# Autodesk Inventor assembly: 二連趕
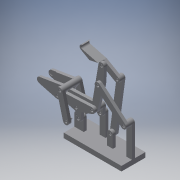
[picture p0: Inventor's stored thumbnail of the model, 180x180]
Saved by Autodesk Inventor 2017 (Build 210142000, 142)
## iProperties
Part Number: 二連趕
Material: 一般
Document SubType Name: Assembly
Designer: 士正
Author: 士正
## Documents named in this file (12)
- C:\Users\士正\Desktop\git\兩段式機構 Inventor版本\二連趕.iam
- C:\Users\士正\Desktop\git\兩段式機構 Inventor版本\實體2.ipt
- C:\Users\士正\Desktop\git\兩段式機構 Inventor版本\實體1.ipt
- C:\Users\士正\Desktop\git\兩段式機構 Inventor版本\實體3.ipt
- C:\Users\士正\Desktop\git\兩段式機構 Inventor版本\實體4.ipt
- C:\Users\士正\Desktop\git\兩段式機構 Inventor版本\實體5.ipt
- C:\Users\士正\Desktop\git\兩段式機構 Inventor版本\實體6.ipt
- C:\Users\士正\Desktop\git\兩段式機構 Inventor版本\實體7.ipt
- C:\Users\士正\Desktop\git\兩段式機構 Inventor版本\實體8.ipt
- C:\Users\士正\Desktop\git\兩段式機構 Inventor版本\實體9.ipt
- C:\Users\士正\Desktop\git\兩段式機構 Inventor版本\實體11.ipt
- C:\Users\士正\Desktop\git\兩段式機構 Inventor版本\pin.ipt
## Components (26 placed, 11 different names)
1. 實體2:1 — 貼合:6, 貼合:15, 貼合:26, 貼合:41, 齊平:11, 貼合:43, 齊平:13
2. 實體1:1 — 貼合:3, 貼合:8, 貼合:21, 貼合:39, 齊平:9, 貼合:60
3. 實體4:1 — 貼合:9, 貼合:11, 貼合:30, 貼合:31
4. 實體5:1 — 貼合:10, 貼合:11, 貼合:31, 貼合:35, 齊平:5
5. 實體6:1 — 貼合:4, 貼合:7, 貼合:33, 齊平:3, 貼合:47, 齊平:18
6. 實體9:1 — 貼合:7, 貼合:8, 貼合:10, 貼合:36, 齊平:6, 貼合:37, 貼合:47, 貼合:60, 貼合:70, 貼合:71
7. 實體11:1 — 貼合:1, 齊平:1, 齊平:2, 貼合:3, 貼合:4, 貼合:6, 貼合:9, 貼合:16, 貼合:21, 貼合:30, 貼合:34, 齊平:4, 貼合:48, 貼合:53, 貼合:58
8. 實體2:2 — 貼合:16, 貼合:53, 貼合:64, 齊平:20, 貼合:66, 貼合:67, 齊平:22, 貼合:68
9. 實體7:2 — 貼合:15, 貼合:26, 貼合:44, 齊平:14, 貼合:56, 貼合:65, 齊平:21, 貼合:66, 貼合:68, 貼合:69
10. pin:1 — 貼合:37, 齊平:18
11. pin:2 — 齊平:17, 貼合:72, 齊平:23
12. pin:3 — 貼合:36, 齊平:6
13. pin:5 — 貼合:67, 齊平:22
14. pin:6 — 貼合:49, 齊平:16
15. pin:7 — 貼合:41, 齊平:11
16. pin:8 — 貼合:35, 齊平:5
17. pin:9 — 貼合:34, 齊平:4
18. pin:10 — 貼合:33, 齊平:3
19. pin:11 — 貼合:39, 齊平:9
20. pin:12
21. pin:13 — 貼合:43, 齊平:13
22. pin:14 — 貼合:44, 齊平:14
23. 實體3:1 — 貼合:48, 貼合:49, 貼合:51, 貼合:55, 貼合:58
24. 實體8:1 — 貼合:51, 貼合:55, 貼合:56, 齊平:16, 齊平:17, 貼合:69, 貼合:70, 貼合:71, 貼合:72, 齊平:23
25. pin:15 — 貼合:65, 齊平:21
26. pin:16 — 貼合:64, 齊平:20
## Relationships (59: Mate 42, Flush 17)
- 貼合:1 [Mate]: 實體11:1
- 齊平:1 [Flush]: 實體11:1
- 齊平:2 [Flush]: 實體11:1
- 貼合:3 [Mate]: 實體1:1 ↔ 實體11:1
- 貼合:4 [Mate]: 實體6:1 ↔ 實體11:1
- 貼合:6 [Mate]: 實體2:1 ↔ 實體11:1
- 貼合:7 [Mate]: 實體6:1 ↔ 實體9:1
- 貼合:8 [Mate]: 實體1:1 ↔ 實體9:1
- 貼合:9 [Mate]: 實體4:1 ↔ 實體11:1
- 貼合:10 [Mate]: 實體5:1 ↔ 實體9:1
- 貼合:11 [Mate]: 實體4:1 ↔ 實體5:1
- 貼合:15 [Mate]: 實體2:1 ↔ 實體7:2
- 貼合:16 [Mate]: 實體11:1 ↔ 實體2:2
- 貼合:21 [Mate]: 實體1:1 ↔ 實體11:1
- 貼合:26 [Mate]: 實體2:1 ↔ 實體7:2
- 貼合:30 [Mate]: 實體4:1 ↔ 實體11:1
- 貼合:31 [Mate]: 實體4:1 ↔ 實體5:1
- 貼合:33 [Mate]: 實體6:1 ↔ pin:10
- 齊平:3 [Flush]: 實體6:1 ↔ pin:10
- 貼合:34 [Mate]: 實體11:1 ↔ pin:9
- 齊平:4 [Flush]: 實體11:1 ↔ pin:9
- 貼合:35 [Mate]: 實體5:1 ↔ pin:8
- 齊平:5 [Flush]: 實體5:1 ↔ pin:8
- 貼合:36 [Mate]: 實體9:1 ↔ pin:3
- 齊平:6 [Flush]: 實體9:1 ↔ pin:3
- 貼合:37 [Mate]: 實體9:1 ↔ pin:1
- 貼合:39 [Mate]: 實體1:1 ↔ pin:11
- 齊平:9 [Flush]: 實體1:1 ↔ pin:11
- 貼合:41 [Mate]: 實體2:1 ↔ pin:7
- 齊平:11 [Flush]: 實體2:1 ↔ pin:7
- 貼合:43 [Mate]: 實體2:1 ↔ pin:13
- 齊平:13 [Flush]: 實體2:1 ↔ pin:13
- 貼合:44 [Mate]: 實體7:2 ↔ pin:14
- 齊平:14 [Flush]: 實體7:2 ↔ pin:14
- 貼合:47 [Mate]: 實體6:1 ↔ 實體9:1
- 貼合:48 [Mate]: 實體11:1 ↔ 實體3:1
- 貼合:49 [Mate]: pin:6 ↔ 實體3:1
- 貼合:51 [Mate]: 實體3:1 ↔ 實體8:1
- 貼合:53 [Mate]: 實體11:1 ↔ 實體2:2
- 貼合:55 [Mate]: 實體3:1 ↔ 實體8:1
- 貼合:56 [Mate]: 實體7:2 ↔ 實體8:1
- 貼合:58 [Mate]: 實體11:1 ↔ 實體3:1
- 貼合:60 [Mate]: 實體1:1 ↔ 實體9:1
- 齊平:16 [Flush]: pin:6 ↔ 實體8:1
- 齊平:17 [Flush]: pin:2 ↔ 實體8:1
- 齊平:18 [Flush]: 實體6:1 ↔ pin:1
- 貼合:64 [Mate]: 實體2:2 ↔ pin:16
- 齊平:20 [Flush]: 實體2:2 ↔ pin:16
- 貼合:65 [Mate]: 實體7:2 ↔ pin:15
- 齊平:21 [Flush]: 實體7:2 ↔ pin:15
- 貼合:66 [Mate]: 實體2:2 ↔ 實體7:2
- 貼合:67 [Mate]: 實體2:2 ↔ pin:5
- 齊平:22 [Flush]: 實體2:2 ↔ pin:5
- 貼合:68 [Mate]: 實體2:2 ↔ 實體7:2
- 貼合:69 [Mate]: 實體7:2 ↔ 實體8:1
- 貼合:70 [Mate]: 實體9:1 ↔ 實體8:1
- 貼合:71 [Mate]: 實體9:1 ↔ 實體8:1
- 貼合:72 [Mate]: pin:2 ↔ 實體8:1
- 齊平:23 [Flush]: pin:2 ↔ 實體8:1
